# Autodesk Inventor assembly: Randverbinder
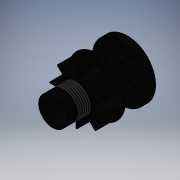
[picture p0: Inventor's stored thumbnail of the model, 180x180]
Saved by Autodesk Inventor 2019 (Build 230136000, 136)
## iProperties
Created: 2019-05-02
Part Number: Randverbinder
Material: Generisch
Document SubType Name: Assembly
Designer: seele
Author: seele
## Documents named in this file (3)
- I:\Desktop\Neuer Ordner\Randverbinder.iam
- I:\Desktop\Neuer Ordner\Randverbinder1.ipt
- I:\Desktop\Neuer Ordner\Randverbinder2.ipt
## Components (2 placed, 2 different names)
1. Randverbinder1:1 — Passend:1, Passend:2, Passend:3, Passend:4, Passend:5, Passend:6, Fluchtend:1
2. Randverbinder2:1 — Passend:1, Passend:2
## Relationships (7: Mate 6, Flush 1)
- Passend:1 [Mate]: Randverbinder1:1 ↔ Randverbinder2:1
- Passend:2 [Mate] (32 mm): Randverbinder1:1 ↔ Randverbinder2:1
- Passend:3 [Mate]: Randverbinder1:1
- Passend:4 [Mate]: Randverbinder1:1
- Passend:5 [Mate]: Randverbinder1:1
- Passend:6 [Mate]: Randverbinder1:1
- Fluchtend:1 [Flush] (-130 mm): Randverbinder1:1
